# Autodesk Inventor assembly: 3x26BoltWasher
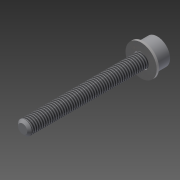
[picture p0: Inventor's stored thumbnail of the model, 180x180]
Saved by Autodesk Inventor 2015 (Build 190159000, 159)
## iProperties
Created: 2014-02-08
Part Number: 3x26BoltWasher
Document SubType Name: Assembly
Designer: Jack
Author: Jack
## Documents named in this file (3)
- C:\Users\Jack\Sync\MendelMax1.5\InventorParts\Hardware\BoltWashers\3x26BoltWasher.iam
- C:\Users\Jack\Sync\MendelMax1.5\InventorParts\Hardware\Bolts\M3x26SHCS.ipt
- C:\Users\Jack\Sync\MendelMax1.5\InventorParts\Hardware\Washers\M3Washer.ipt
## Components (2 placed, 2 different names)
1. M3x26SHCS:1 — Mate:1, Mate:2
2. M3Washer:1 — Mate:1, Mate:2
## Relationships (2: Mate 2)
- Mate:1: M3x26SHCS:1 ↔ M3Washer:1
- Mate:2: M3x26SHCS:1 ↔ M3Washer:1
